# Autodesk Inventor assembly: CellScopeLedArrayAssembly
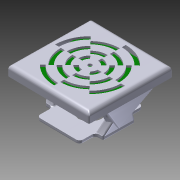
[picture p0: Inventor's stored thumbnail of the model, 180x180]
Saved by Autodesk Inventor 2015 (Build 190159000, 159)
## iProperties
Created: 2015-03-24
Part Number: CellScopeLedArrayAssembly
Document SubType Name: Assembly
Designer: Nitin
Author: Nitin
## Documents named in this file (4)
- C:\Users\Nitin\Documents\CAD Models\CellScopeLedArrayAssembly.iam
- C:\Users\Nitin\Documents\CAD Models\CompCellScopeArrayStage.ipt
- C:\Users\Nitin\Documents\CAD Models\CompCellScopeArray.ipt
- C:\Users\Nitin\Documents\CAD Models\CompCellScopeArrayCover.ipt
## Components (3 placed, 3 different names)
1. CompCellScopeArrayStage:1 — Mate:1, Mate:2, Mate:3, Mate:4, Mate:5, Mate:6, Mate:7, Mate:8, Mate:9
2. CompCellScopeArray:1 — Mate:1, Mate:2, Mate:3, Mate:4, Mate:5
3. CompCellScopeArrayCover:1 — Mate:6, Mate:7, Mate:8, Mate:9
## Relationships (9: Mate 9)
- Mate:1: CompCellScopeArrayStage:1 ↔ CompCellScopeArray:1
- Mate:2: CompCellScopeArrayStage:1 ↔ CompCellScopeArray:1
- Mate:3: CompCellScopeArrayStage:1 ↔ CompCellScopeArray:1
- Mate:4: CompCellScopeArrayStage:1 ↔ CompCellScopeArray:1
- Mate:5: CompCellScopeArrayStage:1 ↔ CompCellScopeArray:1
- Mate:6: CompCellScopeArrayStage:1 ↔ CompCellScopeArrayCover:1
- Mate:7: CompCellScopeArrayStage:1 ↔ CompCellScopeArrayCover:1
- Mate:8: CompCellScopeArrayStage:1 ↔ CompCellScopeArrayCover:1
- Mate:9: CompCellScopeArrayStage:1 ↔ CompCellScopeArrayCover:1
